# Autodesk Inventor assembly: splitter_all
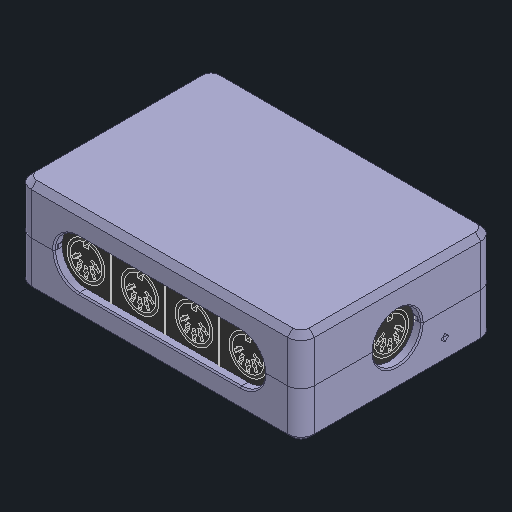
[picture p0: Inventor's stored thumbnail of the model, 512x512]
Saved by Autodesk Inventor 2026.2 (Build 302298000, 298)
## iProperties
Created: 2025-10-04
Part Number: splitter_all
Document SubType Name: Assembly
Designer: micyg
Author: micyg
## Documents named in this file (6)
- D:\Projects\AnotherMidiSplitterV2\Mechanical\splitter_all.iam
- D:\Projects\AnotherMidiSplitterV2\Mechanical\case2.ipt
- D:\Projects\AnotherMidiSplitterV2\Mechanical\mounting.ipt
- D:\Projects\AnotherMidiSplitterV2\Mechanical\case1.ipt
- D:\Projects\AnotherMidiSplitterV2\Mechanical\screw.ipt
- D:\Projects\AnotherMidiSplitterV2\Mechanical\Boards\AnotherMidiSplitterV2_3_0_0\AnotherMidiSplitterV2_v3_0_0\AnotherMidiSplitterV2_v3_0_0\AnotherMidiSplitterV2_v3_0_0.iam
## Components (8 placed, 5 different names)
1. case1:1 — Mate:14, Mate:16, Mate:17, Mate:18, Mate:19, Mate:20
2. case2:1 — Mate:1, Mate:2, Mate:3, Mate:4, Mate:5, Mate:6, Mate:7, Mate:8, Mate:14
3. mounting:1 — Mate:1, Mate:2
4. mounting:2 — Mate:5, Mate:6, Mate:15
5. mounting:3 — Mate:4, Mate:8
6. mounting:4 — Mate:3, Mate:7, Mate:20
7. screw:1 — Mate:15, Mate:16
8. AnotherMidiSplitterV2_v3_0_0:1 [sub-assembly] — Mate:17, Mate:18, Mate:19
## Relationships (15: Mate 15)
- Mate:1: case2:1 ↔ mounting:1
- Mate:2: case2:1 ↔ mounting:1
- Mate:3: case2:1 ↔ mounting:4
- Mate:4: case2:1 ↔ mounting:3
- Mate:5: case2:1 ↔ mounting:2
- Mate:6: case2:1 ↔ mounting:2
- Mate:7: case2:1 ↔ mounting:4
- Mate:8: case2:1 ↔ mounting:3
- Mate:14: case1:1 ↔ case2:1
- Mate:15: mounting:2 ↔ screw:1
- Mate:16: case1:1 ↔ screw:1
- Mate:17: case1:1 ↔ AnotherMidiSplitterV2_v3_0_0:1
- Mate:18: case1:1 ↔ AnotherMidiSplitterV2_v3_0_0:1
- Mate:19: case1:1 ↔ AnotherMidiSplitterV2_v3_0_0:1
- Mate:20: case1:1 ↔ mounting:4
